# Autodesk Inventor assembly: Escritorio2
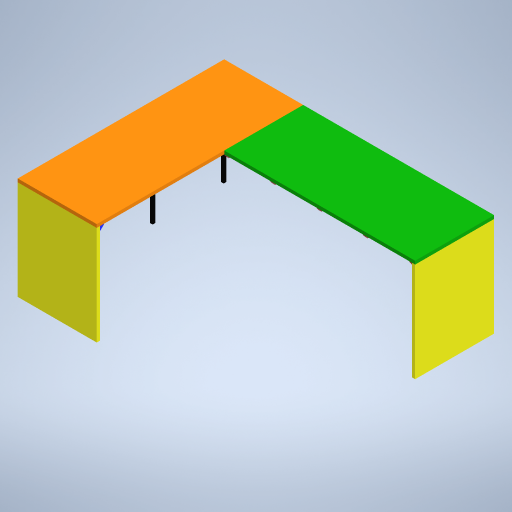
[picture p0: Inventor's stored thumbnail of the model, 512x512]
Saved by Autodesk Inventor 2024 (Build 280153000, 153)
## iProperties
Created: 2023-07-06
Part Number: Escritorio2
Document SubType Name: Assembly
Designer: sergi
Author: sergi
## Documents named in this file (16)
- C:\Users\sergi\OneDrive\Escritorio\proyectos\Escritorio Piso\Escritorio2\Escritorio2.iam
- C:\Users\sergi\OneDrive\Escritorio\proyectos\Escritorio Piso\Escritorio2\Tapa 1.ipt
- C:\Users\sergi\OneDrive\Escritorio\proyectos\Escritorio Piso\Escritorio2\Tapa 2.ipt
- C:\Users\sergi\OneDrive\Escritorio\proyectos\Escritorio Piso\Escritorio2\PataMadera1.ipt
- C:\Users\sergi\OneDrive\Escritorio\proyectos\Escritorio Piso\Escritorio2\Madera Inferior1.ipt
- C:\Users\sergi\OneDrive\Escritorio\proyectos\Escritorio Piso\Escritorio2\Madera Inferior 2.ipt
- C:\Users\sergi\OneDrive\Escritorio\proyectos\Escritorio Piso\BarraLarga.ipt
- C:\Users\sergi\OneDrive\Escritorio\proyectos\Escritorio Piso\Escritorio2\Patas.ipt
- C:\Users\sergi\OneDrive\Escritorio\proyectos\Escritorio Piso\Escritorio2\Union.ipt
- C:\Users\sergi\OneDrive\Escritorio\proyectos\Escritorio Piso\Escritorio2\UnionU.ipt
- C:\Users\sergi\OneDrive\Escritorio\proyectos\Escritorio Piso\Escritorio2\Uniont.ipt
- C:\Users\sergi\OneDrive\Escritorio\proyectos\Escritorio Piso\Escritorio2\UnionU_CPY.ipt
- C:\Users\sergi\OneDrive\Escritorio\proyectos\Escritorio Piso\Escritorio2\UnionV.ipt
- C:\Users\sergi\OneDrive\Escritorio\proyectos\Escritorio Piso\Escritorio2\UnionU_CPY1.ipt
- C:\Users\sergi\OneDrive\Escritorio\STLEscritorio\COTAS.ipt
- C:\Users\sergi\OneDrive\Escritorio\STLEscritorio\bOCETO2.ipt
## Components (44 placed, 15 different names)
1. Tapa 1:1 — Nivelación:1, Coincidencia:1, Nivelación:2, Coincidencia:2, Nivelación:3, Nivelación:4, Nivelación:31, Coincidencia:17, Coincidencia:108, Coincidencia:111, Coincidencia:123, Coincidencia:124
2. Tapa 2:1 — Nivelación:1, Coincidencia:1, Nivelación:2, Coincidencia:3, Nivelación:5, Nivelación:6, Nivelación:11, Coincidencia:7, Coincidencia:9, Nivelación:12, Coincidencia:35, Coincidencia:37, Coincidencia:128, Nivelación:116, Nivelación:117, Nivelación:118, Coincidencia:131, Nivelación:119, Coincidencia:136, Nivelación:126, Coincidencia:138, Coincidencia:143
3. PataMadera1:1 — Coincidencia:2, Nivelación:3, Nivelación:4, Coincidencia:4, Nivelación:7, Nivelación:8, Coincidencia:16, Coincidencia:102
4. PataMadera1:2 — Coincidencia:3, Nivelación:5, Nivelación:6, Coincidencia:5, Nivelación:9, Nivelación:10, Coincidencia:6, Coincidencia:8, Nivelación:13, Nivelación:16, Coincidencia:34, Coincidencia:36, Coincidencia:85, Coincidencia:104, Coincidencia:132
5. Madera Inferior1:1 — Coincidencia:4, Nivelación:7, Nivelación:8, Nivelación:75, Nivelación:95, Nivelación:96, Coincidencia:89, Nivelación:97, Coincidencia:91, Coincidencia:94, Nivelación:98, Nivelación:99, Coincidencia:97, Coincidencia:100, Coincidencia:103, Nivelación:100
6. Madera Inferior 2:1 — Coincidencia:5, Nivelación:9, Nivelación:10, Coincidencia:84, Nivelación:90, Coincidencia:105
7. BarraLarga:1 — Coincidencia:6, Nivelación:11, Coincidencia:7, Nivelación:14, Nivelación:15, Coincidencia:109, Coincidencia:114, Coincidencia:139
8. BarraLarga:2 — Coincidencia:8, Coincidencia:9, Nivelación:12, Nivelación:17, Nivelación:18, Coincidencia:125, Coincidencia:129, Coincidencia:133, Coincidencia:144
9. Patas:1 — Nivelación:13, Nivelación:14, Nivelación:15, Coincidencia:90, Coincidencia:92, Coincidencia:107, Coincidencia:110
10. Patas:2 — Nivelación:16, Nivelación:17, Nivelación:18, Coincidencia:95, Coincidencia:96, Coincidencia:99
11. Union:5 — Nivelación:31, Coincidencia:17
12. Union:6
13. Union:7 — Coincidencia:16
14. Union:8
15. Union:21 — Coincidencia:35, Coincidencia:36
16. Union:22 — Coincidencia:34, Coincidencia:37
17. Union:38 — Nivelación:71, Nivelación:74, Nivelación:75
18. Union:40 — Nivelación:71, Nivelación:74, Coincidencia:101
19. Union:49 — Coincidencia:85
20. Union:50 — Coincidencia:84, Nivelación:90, Coincidencia:106
21. UnionU:1 — Nivelación:95, Nivelación:96, Coincidencia:107, Nivelación:100
22. UnionU:2 — Coincidencia:89, Coincidencia:90, Nivelación:97, Coincidencia:93
23. UnionU:3 — Coincidencia:91, Coincidencia:92, Coincidencia:93
24. Uniont:1 — Coincidencia:94, Nivelación:98, Coincidencia:95
25. Uniont:2 — Nivelación:99, Coincidencia:96, Coincidencia:97, Coincidencia:98
26. Uniont:3 — Coincidencia:98, Coincidencia:99, Coincidencia:100
27. Union:53 — Coincidencia:101, Coincidencia:102, Coincidencia:103
28. Union:54 — Coincidencia:104, Coincidencia:105, Coincidencia:106
29. UnionU:4 — Coincidencia:108, Coincidencia:109, Coincidencia:110, Nivelación:114
30. UnionU:5 — Coincidencia:111, Coincidencia:114, Coincidencia:145
31. UnionU_CPY:1 — Nivelación:108, Nivelación:109, Coincidencia:121, Coincidencia:123, Coincidencia:124, Nivelación:114, Coincidencia:125
32. UnionU_CPY:2 — Nivelación:108, Nivelación:109, Coincidencia:121
33. UnionU_CPY:4 — Coincidencia:128, Coincidencia:129
34. UnionV:1 — Nivelación:116, Nivelación:117, Nivelación:118
35. UnionV:2 — Coincidencia:131, Coincidencia:132, Coincidencia:133, Nivelación:119
36. UnionU_CPY1:1 — Nivelación:120, Nivelación:121, Coincidencia:134, Coincidencia:136, Nivelación:126, Coincidencia:145
37. UnionU_CPY1:2 — Nivelación:120, Nivelación:121, Coincidencia:134, Nivelación:122, Nivelación:124, Coincidencia:135, Nivelación:131
38. UnionU_CPY1:4 — Nivelación:122, Nivelación:124, Coincidencia:135, Coincidencia:140
39. UnionU_CPY1:5 — Coincidencia:138, Coincidencia:139, Coincidencia:140
40. UnionU:12 — Coincidencia:143, Nivelación:131, Coincidencia:144
41. UnionU:13
42. UnionU:14
43. COTAS:1
44. bOCETO2:1
## Relationships (121: Mate 67, Flush 54)
- Nivelación:1 [Flush]: Tapa 1:1 ↔ Tapa 2:1
- Coincidencia:1 [Mate]: Tapa 1:1 ↔ Tapa 2:1
- Nivelación:2 [Flush]: Tapa 1:1 ↔ Tapa 2:1
- Coincidencia:2 [Mate]: Tapa 1:1 ↔ PataMadera1:1
- Nivelación:3 [Flush]: Tapa 1:1 ↔ PataMadera1:1
- Nivelación:4 [Flush]: Tapa 1:1 ↔ PataMadera1:1
- Coincidencia:3 [Mate]: Tapa 2:1 ↔ PataMadera1:2
- Nivelación:5 [Flush]: Tapa 2:1 ↔ PataMadera1:2
- Nivelación:6 [Flush]: Tapa 2:1 ↔ PataMadera1:2
- Coincidencia:4 [Mate]: PataMadera1:1 ↔ Madera Inferior1:1
- Nivelación:7 [Flush] (250 mm): PataMadera1:1 ↔ Madera Inferior1:1
- Nivelación:8 [Flush]: PataMadera1:1 ↔ Madera Inferior1:1
- Coincidencia:5 [Mate]: PataMadera1:2 ↔ Madera Inferior 2:1
- Nivelación:9 [Flush]: PataMadera1:2 ↔ Madera Inferior 2:1
- Nivelación:10 [Flush] (-250 mm): PataMadera1:2 ↔ Madera Inferior 2:1
- Coincidencia:6 [Mate]: PataMadera1:2 ↔ BarraLarga:1
- Nivelación:11 [Flush] (20 mm): Tapa 2:1 ↔ BarraLarga:1
- Coincidencia:7 [Mate]: Tapa 2:1 ↔ BarraLarga:1
- Coincidencia:8 [Mate]: PataMadera1:2 ↔ BarraLarga:2
- Coincidencia:9 [Mate]: Tapa 2:1 ↔ BarraLarga:2
- Nivelación:12 [Flush] (20 mm): Tapa 2:1 ↔ BarraLarga:2
- Nivelación:13 [Flush]: PataMadera1:2 ↔ Patas:1
- Nivelación:14 [Flush]: BarraLarga:1 ↔ Patas:1
- Nivelación:15 [Flush]: BarraLarga:1 ↔ Patas:1
- Nivelación:16 [Flush]: PataMadera1:2 ↔ Patas:2
- Nivelación:17 [Flush]: BarraLarga:2 ↔ Patas:2
- Nivelación:18 [Flush]: BarraLarga:2 ↔ Patas:2
- [Flush]: Union:5 ↔ Union:6
- [Flush]: Union:6 ↔ Union:7
- [Flush]: Union:6 ↔ Union:7
- [Flush]: Union:5 ↔ Union:6
- [Flush]: Union:7 ↔ Union:8
- [Flush]: Union:7 ↔ Union:8
- [Mate] (153.7 mm): Union:5 ↔ Union:8
- [Mate] (153.7 mm): Union:6 ↔ Union:8
- [Mate] (153.7 mm): Union:6 ↔ Union:7
- Coincidencia:16 [Mate]: PataMadera1:1 ↔ Union:7
- Nivelación:31 [Flush]: Tapa 1:1 ↔ Union:5
- Coincidencia:17 [Mate]: Tapa 1:1 ↔ Union:5
- [Mate] (153.7 mm): Union:21 ↔ Union:22
- Coincidencia:34 [Mate]: PataMadera1:2 ↔ Union:22
- Coincidencia:35 [Mate]: Tapa 2:1 ↔ Union:21
- Coincidencia:36 [Mate]: PataMadera1:2 ↔ Union:21
- Coincidencia:37 [Mate]: Tapa 2:1 ↔ Union:22
- [Mate] (230 mm): Union:38 ↔ Union:40
- Nivelación:71 [Flush]: Union:38 ↔ Union:40
- Nivelación:74 [Flush]: Union:38 ↔ Union:40
- Nivelación:75 [Flush]: Madera Inferior1:1 ↔ Union:38
- [Mate] (230 mm): Union:49 ↔ Union:50
- [Flush]: Union:49 ↔ Union:50
- [Flush]: Union:49 ↔ Union:50
- Coincidencia:84 [Mate]: Madera Inferior 2:1 ↔ Union:50
- Coincidencia:85 [Mate]: PataMadera1:2 ↔ Union:49
- Nivelación:90 [Flush]: Madera Inferior 2:1 ↔ Union:50
- Nivelación:95 [Flush]: Madera Inferior1:1 ↔ UnionU:1
- Nivelación:96 [Flush]: Madera Inferior1:1 ↔ UnionU:1
- Coincidencia:89 [Mate]: Madera Inferior1:1 ↔ UnionU:2
- Coincidencia:90 [Mate] (0.5 mm): Patas:1 ↔ UnionU:2
- Nivelación:97 [Flush]: Madera Inferior1:1 ↔ UnionU:2
- Coincidencia:91 [Mate]: Madera Inferior1:1 ↔ UnionU:3
- Coincidencia:92 [Mate] (0.5 mm): Patas:1 ↔ UnionU:3
- Coincidencia:93 [Mate] (115 mm): UnionU:2 ↔ UnionU:3
- Coincidencia:94 [Mate]: Madera Inferior1:1 ↔ Uniont:1
- Nivelación:98 [Flush]: Madera Inferior1:1 ↔ Uniont:1
- Coincidencia:95 [Mate] (0.5 mm): Patas:2 ↔ Uniont:1
- Nivelación:99 [Flush]: Madera Inferior1:1 ↔ Uniont:2
- Coincidencia:96 [Mate] (0.5 mm): Patas:2 ↔ Uniont:2
- Coincidencia:97 [Mate]: Madera Inferior1:1 ↔ Uniont:2
- Coincidencia:98 [Mate] (115 mm): Uniont:2 ↔ Uniont:3
- Coincidencia:99 [Mate] (0.5 mm): Patas:2 ↔ Uniont:3
- Coincidencia:100 [Mate]: Madera Inferior1:1 ↔ Uniont:3
- Coincidencia:101 [Mate] (100 mm): Union:40 ↔ Union:53
- Coincidencia:102 [Mate]: PataMadera1:1 ↔ Union:53
- Coincidencia:103 [Mate]: Madera Inferior1:1 ↔ Union:53
- Coincidencia:104 [Mate]: PataMadera1:2 ↔ Union:54
- Coincidencia:105 [Mate]: Madera Inferior 2:1 ↔ Union:54
- Coincidencia:106 [Mate] (100 mm): Union:50 ↔ Union:54
- Coincidencia:107 [Mate] (0.5 mm): Patas:1 ↔ UnionU:1
- Nivelación:100 [Flush]: Madera Inferior1:1 ↔ UnionU:1
- Coincidencia:108 [Mate]: Tapa 1:1 ↔ UnionU:4
- Coincidencia:109 [Mate] (0.5 mm): BarraLarga:1 ↔ UnionU:4
- Coincidencia:110 [Mate] (5 mm): Patas:1 ↔ UnionU:4
- Coincidencia:111 [Mate]: Tapa 1:1 ↔ UnionU:5
- Coincidencia:114 [Mate] (0.5 mm): BarraLarga:1 ↔ UnionU:5
- Nivelación:108 [Flush]: UnionU_CPY:1 ↔ UnionU_CPY:2
- Nivelación:109 [Flush]: UnionU_CPY:1 ↔ UnionU_CPY:2
- Coincidencia:121 [Mate] (247.5 mm): UnionU_CPY:1 ↔ UnionU_CPY:2
- Coincidencia:123 [Mate]: Tapa 1:1 ↔ UnionU_CPY:1
- Coincidencia:124 [Mate]: Tapa 1:1 ↔ UnionU_CPY:1
- Nivelación:114 [Flush]: UnionU:4 ↔ UnionU_CPY:1
- Coincidencia:125 [Mate] (0.5 mm): BarraLarga:2 ↔ UnionU_CPY:1
- Coincidencia:128 [Mate]: Tapa 2:1 ↔ UnionU_CPY:4
- Coincidencia:129 [Mate] (0.5 mm): BarraLarga:2 ↔ UnionU_CPY:4
- Nivelación:116 [Flush]: Tapa 2:1 ↔ UnionV:1
- Nivelación:117 [Flush]: Tapa 2:1 ↔ UnionV:1
- Nivelación:118 [Flush]: Tapa 2:1 ↔ UnionV:1
- Coincidencia:131 [Mate]: Tapa 2:1 ↔ UnionV:2
- Coincidencia:132 [Mate]: PataMadera1:2 ↔ UnionV:2
- Coincidencia:133 [Mate] (0.5 mm): BarraLarga:2 ↔ UnionV:2
- Nivelación:119 [Flush]: Tapa 2:1 ↔ UnionV:2
- Nivelación:120 [Flush]: UnionU_CPY1:1 ↔ UnionU_CPY1:2
- Nivelación:121 [Flush]: UnionU_CPY1:1 ↔ UnionU_CPY1:2
- Coincidencia:134 [Mate] (329.5 mm): UnionU_CPY1:1 ↔ UnionU_CPY1:2
- Nivelación:122 [Flush]: UnionU_CPY1:2 ↔ UnionU_CPY1:4
- Nivelación:124 [Flush]: UnionU_CPY1:2 ↔ UnionU_CPY1:4
- Coincidencia:135 [Mate] (329.5 mm): UnionU_CPY1:2 ↔ UnionU_CPY1:4
- Coincidencia:136 [Mate]: Tapa 2:1 ↔ UnionU_CPY1:1
- Nivelación:126 [Flush]: Tapa 2:1 ↔ UnionU_CPY1:1
- Coincidencia:138 [Mate]: Tapa 2:1 ↔ UnionU_CPY1:5
- Coincidencia:139 [Mate]: BarraLarga:1 ↔ UnionU_CPY1:5
- Coincidencia:140 [Mate] (329.5 mm): UnionU_CPY1:4 ↔ UnionU_CPY1:5
- [Mate] (329.5 mm): UnionU:12 ↔ UnionU:13
- [Mate] (329.5 mm): UnionU:13 ↔ UnionU:14
- [Flush]: UnionU:13 ↔ UnionU:14
- [Flush]: UnionU:12 ↔ UnionU:13
- [Flush]: UnionU:13 ↔ UnionU:14
- [Flush]: UnionU:12 ↔ UnionU:13
- Coincidencia:143 [Mate]: Tapa 2:1 ↔ UnionU:12
- Nivelación:131 [Flush]: UnionU_CPY1:2 ↔ UnionU:12
- Coincidencia:144 [Mate] (0.5 mm): BarraLarga:2 ↔ UnionU:12
- Coincidencia:145 [Mate] (229.5 mm): UnionU:5 ↔ UnionU_CPY1:1
## Named parameters: d36_d27 = 0 mm, d37_d28 = 0 mm, d38_d29 = 0 mm, d39_d30 = 0 mm, d40_d31 = 0 mm, d41_d32 = 0 mm, d42_d33 = 153.7 mm, d43_d34 = 153.7 mm, d44_d35 = 153.7 mm, d84_d34 = 153.7 mm, d141_d33 = 230 mm, d175_d169_d141_d33 = 230 mm, d176_d170_d144 = 0 mm, d177_d171_d147 = 0 mm, d301_d251_d249 = 329.5 mm, d302_d252_d250 = 329.5 mm, d303_d254 = 0 mm, d304_d255 = 0 mm, d305_d257 = 0 mm, d306_d258 = 0 mm
